# Autodesk Inventor assembly: Swing_Arm_05
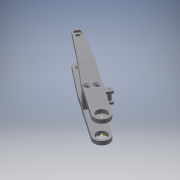
[picture p0: Inventor's stored thumbnail of the model, 180x180]
Saved by Autodesk Inventor 2016 (Build 200138000, 138)
## iProperties
Created: 2016-02-09
Part Number: Swing_Arm_05
Document SubType Name: Assembly
Designer: nils
Author: nils
## Documents named in this file (11)
- D:\bikair\Bikair_CAD-1\Source\Rear_Train\Swing_Arm_05.iam
- D:\bikair\Bikair_CAD-1\Source\Rear_Train\Profile_Straight_05.ipt
- D:\bikair\Bikair_CAD-1\Source\Rear_Train\Profile_Middle_05.ipt
- D:\bikair\Bikair_CAD-1\Source\Rear_Train\Pin_01.ipt
- D:\bikair\Bikair_CAD-1\Source\Rear_Train\Dummy_Plug_01.ipt
- D:\bikair\Bikair_CAD-1\Source\Rear_Train\Swing_Arm_05\AIP\FEA\boqqzixcw.fins
- D:\bikair\Bikair_CAD-1\Source\Rear_Train\Swing_Arm_05\AIP\FEA\boqqzixds.fsat
- D:\bikair\Bikair_CAD-1\Source\Rear_Train\Swing_Arm_05\AIP\FEA\boqqzixds.ftes
- D:\bikair\Bikair_CAD-1\Source\Rear_Train\Swing_Arm_05\AIP\FEA\boqqzixds.fwiz
- D:\bikair\Bikair_CAD-1\Source\Rear_Train\Swing_Arm_05\AIP\FEA\boqqzixk0.fmsh
- D:\bikair\Bikair_CAD-1\Source\Rear_Train\Swing_Arm_05\AIP\FEA\boqqzixk1.fres
## Components (5 placed, 4 different names)
1. Profile_Straight_05:1 — Mate:1, Mate:5, Mate:6
2. Profile_Straight_05:2 — Mate:2, Mate:3, Mate:4
3. Profile_Middle_05:1 — Mate:1, Mate:2, Mate:3, Mate:4, Mate:5, Mate:6, Mate:7, Flush:1, Mate:9
4. Pin_01:1 — Mate:7, Flush:1, Mate:8
5. Dummy_Plug_01:1 — Mate:8, Mate:9
## Relationships (10: Mate 9, Flush 1)
- Mate:1: Profile_Straight_05:1 ↔ Profile_Middle_05:1
- Mate:2: Profile_Straight_05:2 ↔ Profile_Middle_05:1
- Mate:3: Profile_Straight_05:2 ↔ Profile_Middle_05:1
- Mate:4: Profile_Straight_05:2 ↔ Profile_Middle_05:1
- Mate:5: Profile_Straight_05:1 ↔ Profile_Middle_05:1
- Mate:6: Profile_Straight_05:1 ↔ Profile_Middle_05:1
- Mate:7: Profile_Middle_05:1 ↔ Pin_01:1
- Flush:1: Profile_Middle_05:1 ↔ Pin_01:1
- Mate:8: Pin_01:1 ↔ Dummy_Plug_01:1
- Mate:9 (5 mm): Profile_Middle_05:1 ↔ Dummy_Plug_01:1
## Named parameters: sa_0 = 226497, sa_1 = 329696, sa_2 = 1.436e-10, sa_3 = 226497, sa_4 = 329696, sa_5 = 1.14e-10
note: some values were not read from the file. Shown as the stored number, unit unknown: "sa_0", "sa_1", "sa_2", "sa_3", "sa_4", "sa_5".
